# Autodesk Inventor assembly: Assembly
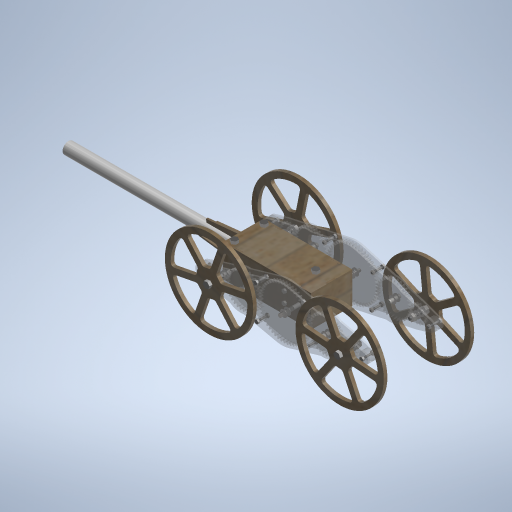
[picture p0: Inventor's stored thumbnail of the model, 512x512]
Saved by Autodesk Inventor 2023 (Build 270158000, 158)
## iProperties
Part Number: Assembly
Document SubType Name: Assembly
Designer: Ronan
Author: Ronan
## Documents named in this file (4)
- D:\Libraries\Documents\2023-FYP\Inventor\Assembly.iam
- D:\Libraries\Documents\2023-FYP\Inventor\LIM.iam
- D:\Libraries\Documents\2023-FYP\Inventor\motor housing.iam
- D:\Libraries\Documents\2023-FYP\Inventor\tail.iam
## Components (4 placed, 3 different names)
1. LIM:1 [sub-assembly] — Cylindrical:1, Mate:2, Tangent:1
2. LIM:2 [sub-assembly] — Cylindrical:2, Mate:1, Tangent:2
3. tail:1 [sub-assembly] — Mate:5, Mate:6, Mate:7
4. motor housing:1 [sub-assembly] — Cylindrical:1, Cylindrical:2, Mate:1, Mate:2, Mate:3, Mate:4, Mate:5, Mate:6, Mate:7, Tangent:1, Tangent:2
## Relationships (11: Mate 7, CylindricalJoint 2, Tangent 2)
- Cylindrical:1: LIM:1 ↔ motor housing:1
- Cylindrical:2: LIM:2 ↔ motor housing:1
- Mate:1: LIM:2 ↔ motor housing:1
- Mate:2: LIM:1 ↔ motor housing:1
- Mate:3: motor housing:1
- Mate:4: motor housing:1
- Mate:5: tail:1 ↔ motor housing:1
- Mate:6: tail:1 ↔ motor housing:1
- Mate:7: tail:1 ↔ motor housing:1
- Tangent:1: LIM:1 ↔ motor housing:1
- Tangent:2: LIM:2 ↔ motor housing:1
